# Autodesk Inventor assembly: Cim Motor Assembly
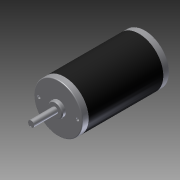
[picture p0: Inventor's stored thumbnail of the model, 180x180]
Saved by Autodesk Inventor 2011 SP1 (Build 150282100, 282)
## iProperties
Created: 2010-12-20
Part Number: Cim Motor Assembly
Document SubType Name: Assembly
Designer: Phillip
Author: Phillip
## Documents named in this file (3)
- C:\Data Folder\FIRST KOP 2011\All Parts 2011\Drive Train\Toughbox\Cim Motor Assembly.iam
- C:\Data Folder\FIRST KOP 2011\All Parts 2011\Drive Train\Toughbox\CIM motor1.ipt
- C:\Data Folder\FIRST KOP 2011\All Parts 2011\Drive Train\Toughbox\CIM Motor Shaft.ipt
## Components (2 placed, 2 different names)
1. CIM motor1:1 — Mate:1, Flush:1
2. CIM Motor Shaft:1 — Mate:1, Flush:1
## Relationships (2: Mate 1, Flush 1)
- Mate:1: CIM motor1:1 ↔ CIM Motor Shaft:1
- Flush:1: CIM motor1:1 ↔ CIM Motor Shaft:1
